# Autodesk Inventor assembly: Carrello semplice
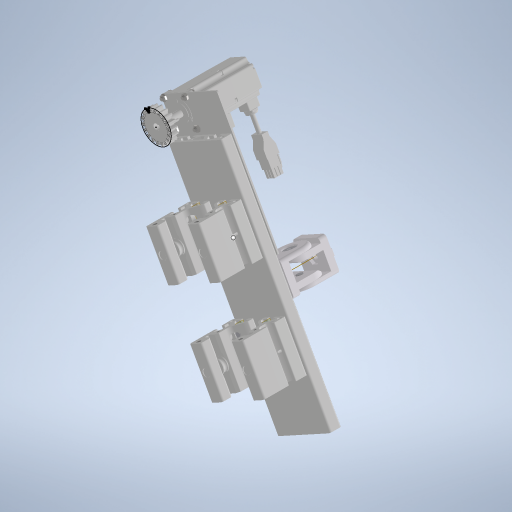
[picture p0: Inventor's stored thumbnail of the model, 512x512]
Saved by Autodesk Inventor 2023 (Build 270158000, 158)
## iProperties
Created: 2021-12-30
Part Number: Carrello semplice
Document SubType Name: Assembly
Designer: matte
Author: matte
## Documents named in this file (15)
- C:\Users\matte\Documents\GitHub\MDM-CyberOrto-CAD\Pezzi singoli\Supporto lineare\Carrello semplice.iam
- C:\Users\matte\Documents\GitHub\MDM-CyberOrto-CAD\Pezzi singoli\Supporto lineare\Piastra-supporto.ipt
- C:\Users\matte\Documents\GitHub\MDM-CyberOrto-CAD\Parker components\08-Linear Application\06-Linear Roller System\01-Roller System 6\30-401.ipt
- C:\Users\matte\Documents\GitHub\MDM-CyberOrto-CAD\Pezzi singoli\Supporto lineare\Doppia Giuntura.iam
- C:\Users\matte\Documents\GitHub\MDM-CyberOrto-CAD\Parker components\05-Handles_Hinges\13-Pivot Joints\23-010.iam
- C:\Users\matte\Documents\GitHub\MDM-CyberOrto-CAD\Parker components\02-Fasteners\10-Standard T-Nuts\20-058.ipt
- C:\Users\matte\Documents\GitHub\MDM-CyberOrto-CAD\Parker components\02-Fasteners\16-Screws\01-Metric Screws\01-Button Head\24-116-8.ipt
- C:\Users\matte\Documents\GitHub\MDM-CyberOrto-CAD\Rack_Pinion\piastra_motore.ipt
- C:\Users\matte\Documents\GitHub\MDM-CyberOrto-CAD\Servo Motor 50W\bch2mba531ca5c.ipt
- C:\Users\matte\Documents\GitHub\MDM-CyberOrto-CAD\Rack_Pinion\Pinion.ipt
- C:\Users\matte\Documents\GitHub\MDM-CyberOrto-CAD\Inventor Support\Content Center Files\it-IT\AS 1474(1)\AS 1474 - M4(1).ipt
- C:\Users\matte\Documents\GitHub\MDM-CyberOrto-CAD\Inventor Support\Content Center Files\it-IT\ISO 1580\ISO 1580 - M4 x 12_.ipt
- C:\Users\matte\Documents\GitHub\MDM-CyberOrto-CAD\Parker components\02-Fasteners\10-Standard T-Nuts\20-050.ipt
- C:\Users\matte\Documents\GitHub\MDM-CyberOrto-CAD\Parker components\02-Fasteners\15-T-Bolts_Nuts_Washers\03-Washers\24-708-8.ipt
- C:\Users\matte\Documents\GitHub\MDM-CyberOrto-CAD\Parker components\02-Fasteners\16-Screws\01-Metric Screws\03-Socket Head\24-330-8.ipt
## Components (31 placed, 14 different names)
1. Piastra-supporto:1 — Allineato:7, Coincidente:6, Coincidente:7, Coincidente:11, Coincidente:12, Allineato:20, Allineato:21, Angolo:1, Coincidente:21, Coincidente:24, Coincidente:25, Allineato:22, Coincidente:48, Coincidente:67
2. 30-401:1 — Coincidente:19, Coincidente:56
3. 30-401:2 — Coincidente:24
4. 30-401:3 — Coincidente:68
5. 30-401:4 — Coincidente:8
6. Doppia Giuntura:1 [sub-assembly] — Coincidente:6, Coincidente:7, Coincidente:8, Coincidente:15
7. Doppia Giuntura:2 [sub-assembly] — Coincidente:11, Coincidente:12, Coincidente:15
8. 23-010:1 [sub-assembly] — Allineato:20, Allineato:21, Coincidente:19, Coincidente:20, Coincidente:22, Coincidente:23, Coincidente:26
9. 20-058:1 — Coincidente:20, Angolo:1, Coincidente:21
10. 24-116-8:1 — Coincidente:22, Coincidente:23
11. piastra_motore:1 — Coincidente:25, Coincidente:26, Allineato:22, Coincidente:27, Allineato:23, Allineato:24, Coincidente:43, Coincidente:44, Coincidente:45, Coincidente:46, Coincidente:48, Coincidente:55, Coincidente:63, Coincidente:64, Coincidente:65, Coincidente:66, Coincidente:69, Coincidente:70
12. bch2mba531ca5c:1 — Coincidente:27, Allineato:23, Allineato:24, Coincidente:28, Allineato:25, Coincidente:35, Coincidente:36, Coincidente:37, Coincidente:38, Coincidente:39, Coincidente:40, Coincidente:41, Coincidente:42
13. Pinion:1 — Coincidente:28, Allineato:25
14. 24-330-8:1 — Coincidente:49, Coincidente:50, Coincidente:54, Coincidente:69
15. 20-050:1 — Coincidente:53, Coincidente:54, Coincidente:56
16. 24-708-8:1 — Coincidente:49, Coincidente:50, Allineato:26, Coincidente:55
17. 24-330-8:2 — Coincidente:53, Coincidente:70
18. 24-708-8:2 — Allineato:26
19. 24-330-8:3 — Coincidente:63, Coincidente:65, Coincidente:66
20. 20-050:2 — Coincidente:68
21. 24-708-8:3 — Coincidente:64
22. 24-330-8:4 — Coincidente:67
23. 24-708-8:4
24. AS 1474 - Metrico M4:1 — Coincidente:30, Coincidente:45
25. ISO 1580 M4 x 12:1 — Coincidente:30, Coincidente:35, Coincidente:36
26. AS 1474 - Metrico M4:2 — Coincidente:43
27. ISO 1580 M4 x 12:2 — Coincidente:37, Coincidente:38
28. AS 1474 - Metrico M4:3 — Coincidente:46
29. ISO 1580 M4 x 12:3 — Coincidente:41, Coincidente:42
30. AS 1474 - Metrico M4:4 — Coincidente:44
31. ISO 1580 M4 x 12:4 — Coincidente:39, Coincidente:40
## Relationships (78: Mate 62, Flush 15, Angle 1)
- [Mate]: Piastra-supporto:1 ↔ 30-401:1
- [Flush]: Piastra-supporto:1 ↔ 30-401:1
- [Flush]: Piastra-supporto:1 ↔ 30-401:2
- [Mate]: Piastra-supporto:1 ↔ 30-401:2
- [Mate] (60 mm): 30-401:1 ↔ 30-401:2
- [Mate]: Piastra-supporto:1 ↔ 30-401:3
- [Flush]: Piastra-supporto:1 ↔ 30-401:3
- [Flush]: 30-401:1 ↔ 30-401:3
- [Mate]: Piastra-supporto:1 ↔ 30-401:4
- [Flush]: Piastra-supporto:1 ↔ 30-401:4
- [Flush]: 30-401:2 ↔ 30-401:4
- Allineato:7 [Flush]: Piastra-supporto:1
- Coincidente:6 [Mate]: Piastra-supporto:1 ↔ Doppia Giuntura:1
- Coincidente:7 [Mate]: Piastra-supporto:1 ↔ Doppia Giuntura:1
- Coincidente:8 [Mate]: 30-401:4 ↔ Doppia Giuntura:1
- Coincidente:11 [Mate]: Piastra-supporto:1 ↔ Doppia Giuntura:2
- Coincidente:12 [Mate]: Piastra-supporto:1 ↔ Doppia Giuntura:2
- Coincidente:15 [Mate]: Doppia Giuntura:1 ↔ Doppia Giuntura:2
- Allineato:20 [Flush]: Piastra-supporto:1 ↔ 23-010:1
- Allineato:21 [Flush]: Piastra-supporto:1 ↔ 23-010:1
- Coincidente:19 [Mate] (30 mm): 30-401:1 ↔ 23-010:1
- Coincidente:20 [Mate]: 23-010:1 ↔ 20-058:1
- Angolo:1 [Angle] (0 deg): Piastra-supporto:1 ↔ 20-058:1
- Coincidente:21 [Mate]: Piastra-supporto:1 ↔ 20-058:1
- Coincidente:22 [Mate]: 23-010:1 ↔ 24-116-8:1
- Coincidente:23 [Mate]: 23-010:1 ↔ 24-116-8:1
- Coincidente:24 [Mate] (60 mm): Piastra-supporto:1 ↔ 30-401:2
- Coincidente:25 [Mate]: Piastra-supporto:1 ↔ piastra_motore:1
- Coincidente:26 [Mate] (5 mm): 23-010:1 ↔ piastra_motore:1
- Allineato:22 [Flush]: Piastra-supporto:1 ↔ piastra_motore:1
- Coincidente:27 [Mate]: piastra_motore:1 ↔ bch2mba531ca5c:1
- Allineato:23 [Flush]: piastra_motore:1 ↔ bch2mba531ca5c:1
- Allineato:24 [Flush]: piastra_motore:1 ↔ bch2mba531ca5c:1
- Coincidente:28 [Mate]: bch2mba531ca5c:1 ↔ Pinion:1
- Allineato:25 [Flush] (-10 mm): bch2mba531ca5c:1 ↔ Pinion:1
- [Mate]: AS 1474 - Metrico M4:1 ↔ ISO 1580 M4 x 12:1
- Coincidente:30 [Mate] (7.715 mm): AS 1474 - Metrico M4:1 ↔ ISO 1580 M4 x 12:1
- [Mate]: AS 1474 - Metrico M4:2 ↔ ISO 1580 M4 x 12:2
- [Mate]: AS 1474 - Metrico M4:3 ↔ ISO 1580 M4 x 12:3
- [Mate] (7.715 mm): AS 1474 - Metrico M4:3 ↔ ISO 1580 M4 x 12:3
- [Mate]: AS 1474 - Metrico M4:4 ↔ ISO 1580 M4 x 12:4
- Coincidente:35 [Mate]: bch2mba531ca5c:1 ↔ ISO 1580 M4 x 12:1
- Coincidente:36 [Mate]: bch2mba531ca5c:1 ↔ ISO 1580 M4 x 12:1
- Coincidente:37 [Mate]: bch2mba531ca5c:1 ↔ ISO 1580 M4 x 12:2
- Coincidente:38 [Mate]: bch2mba531ca5c:1 ↔ ISO 1580 M4 x 12:2
- Coincidente:39 [Mate]: bch2mba531ca5c:1 ↔ ISO 1580 M4 x 12:4
- Coincidente:40 [Mate]: bch2mba531ca5c:1 ↔ ISO 1580 M4 x 12:4
- Coincidente:41 [Mate]: bch2mba531ca5c:1 ↔ ISO 1580 M4 x 12:3
- Coincidente:42 [Mate]: bch2mba531ca5c:1 ↔ ISO 1580 M4 x 12:3
- Coincidente:43 [Mate]: piastra_motore:1 ↔ AS 1474 - Metrico M4:2
- Coincidente:44 [Mate]: piastra_motore:1 ↔ AS 1474 - Metrico M4:4
- Coincidente:45 [Mate]: piastra_motore:1 ↔ AS 1474 - Metrico M4:1
- Coincidente:46 [Mate]: piastra_motore:1 ↔ AS 1474 - Metrico M4:3
- Coincidente:48 [Mate]: Piastra-supporto:1 ↔ piastra_motore:1
- Coincidente:49 [Mate]: 24-330-8:1 ↔ 24-708-8:1
- Coincidente:50 [Mate]: 24-330-8:1 ↔ 24-708-8:1
- [Mate]: 24-330-8:2 ↔ 24-708-8:2
- [Mate]: 24-330-8:2 ↔ 24-708-8:2
- Coincidente:53 [Mate]: 20-050:1 ↔ 24-330-8:2
- Coincidente:54 [Mate]: 24-330-8:1 ↔ 20-050:1
- Allineato:26 [Flush]: 24-708-8:1 ↔ 24-708-8:2
- Coincidente:55 [Mate]: piastra_motore:1 ↔ 24-708-8:1
- Coincidente:56 [Mate]: 30-401:1 ↔ 20-050:1
- [Mate]: 24-330-8:3 ↔ 24-708-8:3
- [Mate]: 24-330-8:3 ↔ 24-708-8:3
- [Mate]: 24-330-8:4 ↔ 24-708-8:4
- [Mate]: 24-330-8:4 ↔ 24-708-8:4
- [Mate]: 20-050:2 ↔ 24-330-8:4
- [Mate]: 24-330-8:3 ↔ 20-050:2
- [Flush]: 24-708-8:3 ↔ 24-708-8:4
- Coincidente:63 [Mate]: piastra_motore:1 ↔ 24-330-8:3
- Coincidente:64 [Mate]: piastra_motore:1 ↔ 24-708-8:3
- Coincidente:65 [Mate]: piastra_motore:1 ↔ 24-330-8:3
- Coincidente:66 [Mate]: piastra_motore:1 ↔ 24-330-8:3
- Coincidente:67 [Mate]: Piastra-supporto:1 ↔ 24-330-8:4
- Coincidente:68 [Mate]: 30-401:3 ↔ 20-050:2
- Coincidente:69 [Mate]: piastra_motore:1 ↔ 24-330-8:1
- Coincidente:70 [Mate]: piastra_motore:1 ↔ 24-330-8:2
## Named parameters: d78_d351 = 0 mm, d79_d351 = 0 mm, d80_d77 = 7.715 mm, d81_d78_d351 = 0 mm, d113_d111 = 0 mm, d114_d112 = 0 mm, d120_d115 = 0 mm, d121_d116 = 0 mm, d122_d117 = 0 mm, d123_d111 = 0 mm, d124_d112 = 0 mm, d125_d113_d111 = 0 mm, d126_d114_d112 = 0 mm
